# Autodesk Inventor assembly: arm
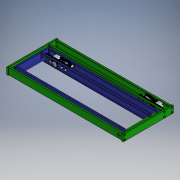
[picture p0: Inventor's stored thumbnail of the model, 180x180]
Saved by Autodesk Inventor 2022 (Build 260153000, 153)
## iProperties
Created: 2021-06-08
Part Number: arm
Document SubType Name: Assembly
Designer: yossy
Mass: 1577.87 g
Surface Area: 2797.55 cm^2
Volume: 584.398 cm^3
Density: 2.7 g/cm^3
Author: yossy
## Documents named in this file (21)
- C:\Users\nrz71\Documents\Inventor\arm\arm.iam
- C:\Users\nrz71\Documents\Inventor\arm\arm1_L.ipt
- C:\Users\nrz71\Documents\Inventor\arm\arm1_S.ipt
- C:\Users\nrz71\Documents\Inventor\arm\arm1_L_hole.ipt
- C:\Users\nrz71\Documents\Inventor\arm\arm1_L_M.ipt
- C:\Users\nrz71\Documents\Inventor\arm\110041_AMAX16_EB_2W_SL_1WE.ipt
- C:\Users\nrz71\Downloads\PARTserver0202107062223180363888451784290\BS2M30.ipt
- C:\Users\nrz71\Documents\Inventor\arm\arm\デザイン アクセラレータ\平歯車3.iam
- C:\Users\nrz71\Documents\Inventor\arm\軸.ipt
- C:\Users\nrz71\Downloads\BS2M14_Autodesk_Inventor_2020_20210707\BS2M14.ipt
- C:\Users\nrz71\Documents\Inventor\arm\arm\デザイン アクセラレータ\平歯車6.iam
- C:\Users\nrz71\Documents\Inventor\arm\大軸.ipt
- C:\Users\nrz71\Documents\Inventor\arm\arm1_L - コピー.ipt
- C:\Users\nrz71\Documents\Inventor\arm\arm1_L_hole - コピー.ipt
- C:\Users\nrz71\Documents\Inventor\arm\arm1_S - コピー.ipt
- C:\Users\nrz71\Documents\Inventor\arm\arm1_L_M - コピー.ipt
- C:\Users\nrz71\Documents\Inventor\arm\中軸.ipt
- C:\Users\nrz71\Documents\Inventor\arm\ベアリング\ベアリング4-7.ipt
- C:\Users\nrz71\Documents\Inventor\arm\ベアリング\ベアリング6-10.ipt
- C:\Users\nrz71\Documents\Inventor\arm\s2m187.ipt
- C:\Users\nrz71\Documents\Inventor\arm\s2m88.ipt
## Components (53 placed, 19 different names)
1. arm1_L:1 — メイト:1, メイト:2, フラッシュ:1, フラッシュ:3, フラッシュ:4, 正接:1, メイト:6, メイト:7, フラッシュ:6, メイト:24, メイト:25, フラッシュ:8, フラッシュ:18, メイト:45, メイト:59, メイト:61, メイト:62, メイト:65, メイト:71, メイト:115
2. arm1_S:1 — メイト:1, メイト:2, フラッシュ:1, メイト:3, フラッシュ:2, メイト:4, フラッシュ:5
3. arm1_L_hole:1 — フラッシュ:3, フラッシュ:4, メイト:5, メイト:10, メイト:11, メイト:13, メイト:17, メイト:22, メイト:23, メイト:27, メイト:28, メイト:29, メイト:31, メイト:32, メイト:39, メイト:47, メイト:48, メイト:58, メイト:63, メイト:64, メイト:70, フラッシュ:24, フラッシュ:25
4. arm1_L_M:1 — メイト:3, フラッシュ:2, メイト:4, メイト:68
5. 110041_AMAX16_EB_2W_SL_1WE:1 — メイト:5, 正接:1, メイト:6, メイト:13, メイト:21
6. arm1_S:2 — フラッシュ:5, メイト:7, フラッシュ:6
7. BS2M30:1 — メイト:10, メイト:11
8. 軸:1 — メイト:17, メイト:20, フラッシュ:18, メイト:57, メイト:60, メイト:116
9. BS2M30:2 — メイト:24, メイト:26, メイト:27
10. BS2M14:1 — メイト:20, メイト:25
11. 平歯車:1 [sub-assembly] — メイト:21, メイト:22, メイト:23
12. 平歯車:2 [sub-assembly] — メイト:26, メイト:28, メイト:30
13. BS2M30:3 — メイト:29, メイト:30, メイト:31
14. 大軸:1 — フラッシュ:8, メイト:32, メイト:33, メイト:66, メイト:67, メイト:69
15. arm1_L - コピー:1 — メイト:33, メイト:34, フラッシュ:10, メイト:35, フラッシュ:11, メイト:37, フラッシュ:12, メイト:38, フラッシュ:16, メイト:42, メイト:49, メイト:50, メイト:55, メイト:56, メイト:75, メイト:80, メイト:81, フラッシュ:22, メイト:90, メイト:97, フラッシュ:24, メイト:114
16. arm1_L_hole - コピー:1 — メイト:34, フラッシュ:10, メイト:36, メイト:51, メイト:52, メイト:53, メイト:54, メイト:77, メイト:78, メイト:79, メイト:99, メイト:110
17. 110041_AMAX16_EB_2W_SL_1WE:2 — メイト:35, フラッシュ:11, メイト:36, メイト:100
18. arm1_S - コピー:1 — メイト:37, フラッシュ:12, メイト:38, メイト:39, メイト:40, メイト:41, フラッシュ:13
19. arm1_L_M - コピー:1 — メイト:40, メイト:41, フラッシュ:13, メイト:72
20. 中軸:1 — フラッシュ:16, メイト:42, メイト:73, メイト:74, メイト:76, メイト:87, メイト:111
21. ベアリング4-7:2 — メイト:59, メイト:60
22. ベアリング4-7:3 — メイト:45, メイト:71, メイト:82, フラッシュ:19
23. ベアリング4-7:4 — メイト:47, メイト:48
24. ベアリング4-7:6 — メイト:49, メイト:50
25. ベアリング4-7:7 — メイト:55, メイト:56, フラッシュ:21
26. ベアリング4-7:8 — メイト:53, メイト:54, メイト:86
27. ベアリング4-7:9 — メイト:51, メイト:52, メイト:85
28. ベアリング4-7:10 — メイト:57, メイト:58
29. ベアリング6-10:1 — メイト:65, メイト:66
30. ベアリング6-10:2 — メイト:67, メイト:68
31. ベアリング6-10:3 — メイト:74, メイト:75
32. ベアリング6-10:4 — メイト:72, メイト:73
33. ベアリング4-7:11 — メイト:63, メイト:64
34. ベアリング4-7:12 — メイト:61, メイト:62, メイト:83, フラッシュ:20
35. ベアリング6-10:5 — メイト:69, メイト:70
36. ベアリング6-10:6 — メイト:76, メイト:77, メイト:92
37. ベアリング4-7:13 — メイト:80, メイト:81, フラッシュ:23
38. ベアリング4-7:14 — メイト:78, メイト:79, メイト:84, メイト:91
39. 軸:2 — メイト:82, フラッシュ:19, メイト:117
40. 軸:3 — メイト:83, フラッシュ:20
41. 軸:4 — メイト:86, フラッシュ:21, メイト:96, メイト:98, メイト:112
42. 軸:5 — メイト:85, フラッシュ:22, メイト:89, メイト:95, メイト:113
43. 軸:6 — メイト:84, フラッシュ:23, メイト:88, メイト:94, メイト:109
44. BS2M30:4 — メイト:87, メイト:92
45. BS2M30:5 — メイト:89, メイト:90
46. BS2M30:6 — メイト:88, メイト:91, メイト:93
47. 平歯車:3 [sub-assembly] — メイト:93, メイト:94, メイト:95
48. BS2M14:2 — メイト:96, メイト:97
49. 平歯車:4 [sub-assembly] — メイト:98, メイト:99, メイト:100
50. s2m187:1 — フラッシュ:25
51. s2m187:2 — メイト:109, メイト:110, メイト:111
52. s2m88:1 — メイト:112, メイト:113, メイト:114
53. s2m88:2 — メイト:115, メイト:116, メイト:117
## Relationships (119: Mate 98, Flush 20, Tangent 1)
- メイト:1 [Mate]: arm1_L:1 ↔ arm1_S:1
- メイト:2 [Mate]: arm1_L:1 ↔ arm1_S:1
- フラッシュ:1 [Flush]: arm1_L:1 ↔ arm1_S:1
- メイト:3 [Mate]: arm1_S:1 ↔ arm1_L_M:1
- フラッシュ:2 [Flush]: arm1_S:1 ↔ arm1_L_M:1
- メイト:4 [Mate]: arm1_S:1 ↔ arm1_L_M:1
- フラッシュ:3 [Flush]: arm1_L:1 ↔ arm1_L_hole:1
- フラッシュ:4 [Flush]: arm1_L:1 ↔ arm1_L_hole:1
- メイト:5 [Mate]: arm1_L_hole:1 ↔ 110041_AMAX16_EB_2W_SL_1WE:1
- 正接:1 [Tangent]: arm1_L:1 ↔ 110041_AMAX16_EB_2W_SL_1WE:1
- メイト:6 [Mate]: arm1_L:1 ↔ 110041_AMAX16_EB_2W_SL_1WE:1
- フラッシュ:5 [Flush]: arm1_S:1 ↔ arm1_S:2
- メイト:7 [Mate]: arm1_L:1 ↔ arm1_S:2
- フラッシュ:6 [Flush]: arm1_L:1 ↔ arm1_S:2
- メイト:10 [Mate]: arm1_L_hole:1 ↔ BS2M30:1
- メイト:11 [Mate]: arm1_L_hole:1 ↔ BS2M30:1
- メイト:13 [Mate]: arm1_L_hole:1 ↔ 110041_AMAX16_EB_2W_SL_1WE:1
- メイト:17 [Mate]: arm1_L_hole:1 ↔ 軸:1
- メイト:20 [Mate]: 軸:1 ↔ BS2M14:1
- メイト:21 [Mate]: 110041_AMAX16_EB_2W_SL_1WE:1 ↔ 平歯車:1
- メイト:22 [Mate]: arm1_L_hole:1 ↔ 平歯車:1
- メイト:23 [Mate]: arm1_L_hole:1 ↔ 平歯車:1
- メイト:24 [Mate]: arm1_L:1 ↔ BS2M30:2
- メイト:25 [Mate]: arm1_L:1 ↔ BS2M14:1
- メイト:26 [Mate]: BS2M30:2 ↔ 平歯車:2
- メイト:27 [Mate]: arm1_L_hole:1 ↔ BS2M30:2
- メイト:28 [Mate]: arm1_L_hole:1 ↔ 平歯車:2
- メイト:29 [Mate]: arm1_L_hole:1 ↔ BS2M30:3
- メイト:30 [Mate]: 平歯車:2 ↔ BS2M30:3
- メイト:31 [Mate]: arm1_L_hole:1 ↔ BS2M30:3
- フラッシュ:8 [Flush]: arm1_L:1 ↔ 大軸:1
- メイト:32 [Mate]: arm1_L_hole:1 ↔ 大軸:1
- メイト:33 [Mate]: 大軸:1 ↔ arm1_L - コピー:1
- メイト:34 [Mate]: arm1_L - コピー:1 ↔ arm1_L_hole - コピー:1
- フラッシュ:10 [Flush]: arm1_L - コピー:1 ↔ arm1_L_hole - コピー:1
- メイト:35 [Mate]: arm1_L - コピー:1 ↔ 110041_AMAX16_EB_2W_SL_1WE:2
- フラッシュ:11 [Flush]: arm1_L - コピー:1 ↔ 110041_AMAX16_EB_2W_SL_1WE:2
- メイト:36 [Mate]: arm1_L_hole - コピー:1 ↔ 110041_AMAX16_EB_2W_SL_1WE:2
- メイト:37 [Mate]: arm1_L - コピー:1 ↔ arm1_S - コピー:1
- フラッシュ:12 [Flush]: arm1_L - コピー:1 ↔ arm1_S - コピー:1
- メイト:38 [Mate]: arm1_L - コピー:1 ↔ arm1_S - コピー:1
- メイト:39 [Mate] (3 mm): arm1_L_hole:1 ↔ arm1_S - コピー:1
- メイト:40 [Mate]: arm1_S - コピー:1 ↔ arm1_L_M - コピー:1
- メイト:41 [Mate]: arm1_S - コピー:1 ↔ arm1_L_M - コピー:1
- フラッシュ:13 [Flush]: arm1_S - コピー:1 ↔ arm1_L_M - コピー:1
- フラッシュ:16 [Flush]: arm1_L - コピー:1 ↔ 中軸:1
- メイト:42 [Mate]: arm1_L - コピー:1 ↔ 中軸:1
- フラッシュ:18 [Flush]: arm1_L:1 ↔ 軸:1
- メイト:45 [Mate]: arm1_L:1 ↔ ベアリング4-7:3
- メイト:47 [Mate]: arm1_L_hole:1 ↔ ベアリング4-7:4
- メイト:48 [Mate]: arm1_L_hole:1 ↔ ベアリング4-7:4
- メイト:49 [Mate]: arm1_L - コピー:1 ↔ ベアリング4-7:6
- メイト:50 [Mate]: arm1_L - コピー:1 ↔ ベアリング4-7:6
- メイト:51 [Mate]: arm1_L_hole - コピー:1 ↔ ベアリング4-7:9
- メイト:52 [Mate]: arm1_L_hole - コピー:1 ↔ ベアリング4-7:9
- メイト:53 [Mate]: arm1_L_hole - コピー:1 ↔ ベアリング4-7:8
- メイト:54 [Mate]: arm1_L_hole - コピー:1 ↔ ベアリング4-7:8
- メイト:55 [Mate]: arm1_L - コピー:1 ↔ ベアリング4-7:7
- メイト:56 [Mate]: arm1_L - コピー:1 ↔ ベアリング4-7:7
- メイト:57 [Mate]: 軸:1 ↔ ベアリング4-7:10
- メイト:58 [Mate]: arm1_L_hole:1 ↔ ベアリング4-7:10
- メイト:59 [Mate]: arm1_L:1 ↔ ベアリング4-7:2
- メイト:60 [Mate]: 軸:1 ↔ ベアリング4-7:2
- メイト:61 [Mate]: arm1_L:1 ↔ ベアリング4-7:12
- メイト:62 [Mate]: arm1_L:1 ↔ ベアリング4-7:12
- メイト:63 [Mate]: arm1_L_hole:1 ↔ ベアリング4-7:11
- メイト:64 [Mate]: arm1_L_hole:1 ↔ ベアリング4-7:11
- メイト:65 [Mate]: arm1_L:1 ↔ ベアリング6-10:1
- メイト:66 [Mate]: 大軸:1 ↔ ベアリング6-10:1
- メイト:67 [Mate]: 大軸:1 ↔ ベアリング6-10:2
- メイト:68 [Mate]: arm1_L_M:1 ↔ ベアリング6-10:2
- メイト:69 [Mate]: 大軸:1 ↔ ベアリング6-10:5
- メイト:70 [Mate]: arm1_L_hole:1 ↔ ベアリング6-10:5
- メイト:71 [Mate]: arm1_L:1 ↔ ベアリング4-7:3
- メイト:72 [Mate]: arm1_L_M - コピー:1 ↔ ベアリング6-10:4
- メイト:73 [Mate]: 中軸:1 ↔ ベアリング6-10:4
- メイト:74 [Mate]: 中軸:1 ↔ ベアリング6-10:3
- メイト:75 [Mate]: arm1_L - コピー:1 ↔ ベアリング6-10:3
- メイト:76 [Mate]: 中軸:1 ↔ ベアリング6-10:6
- メイト:77 [Mate]: arm1_L_hole - コピー:1 ↔ ベアリング6-10:6
- メイト:78 [Mate]: arm1_L_hole - コピー:1 ↔ ベアリング4-7:14
- メイト:79 [Mate]: arm1_L_hole - コピー:1 ↔ ベアリング4-7:14
- メイト:80 [Mate]: arm1_L - コピー:1 ↔ ベアリング4-7:13
- メイト:81 [Mate]: arm1_L - コピー:1 ↔ ベアリング4-7:13
- メイト:82 [Mate]: ベアリング4-7:3 ↔ 軸:2
- フラッシュ:19 [Flush]: ベアリング4-7:3 ↔ 軸:2
- メイト:83 [Mate]: ベアリング4-7:12 ↔ 軸:3
- フラッシュ:20 [Flush]: ベアリング4-7:12 ↔ 軸:3
- メイト:84 [Mate]: ベアリング4-7:14 ↔ 軸:6
- メイト:85 [Mate]: ベアリング4-7:9 ↔ 軸:5
- メイト:86 [Mate]: ベアリング4-7:8 ↔ 軸:4
- フラッシュ:21 [Flush]: ベアリング4-7:7 ↔ 軸:4
- フラッシュ:22 [Flush]: arm1_L - コピー:1 ↔ 軸:5
- フラッシュ:23 [Flush]: ベアリング4-7:13 ↔ 軸:6
- メイト:87 [Mate]: 中軸:1 ↔ BS2M30:4
- メイト:88 [Mate]: 軸:6 ↔ BS2M30:6
- メイト:89 [Mate]: 軸:5 ↔ BS2M30:5
- メイト:90 [Mate]: arm1_L - コピー:1 ↔ BS2M30:5
- メイト:91 [Mate]: ベアリング4-7:14 ↔ BS2M30:6
- メイト:92 [Mate]: ベアリング6-10:6 ↔ BS2M30:4
- メイト:93 [Mate]: BS2M30:6 ↔ 平歯車:3
- メイト:94 [Mate]: 軸:6 ↔ 平歯車:3
- メイト:95 [Mate]: 軸:5 ↔ 平歯車:3
- メイト:96 [Mate]: 軸:4 ↔ BS2M14:2
- メイト:97 [Mate]: arm1_L - コピー:1 ↔ BS2M14:2
- メイト:98 [Mate]: 軸:4 ↔ 平歯車:4
- メイト:99 [Mate]: arm1_L_hole - コピー:1 ↔ 平歯車:4
- メイト:100 [Mate]: 110041_AMAX16_EB_2W_SL_1WE:2 ↔ 平歯車:4
- フラッシュ:24 [Flush]: arm1_L_hole:1 ↔ arm1_L - コピー:1
- フラッシュ:25 [Flush]: arm1_L_hole:1 ↔ s2m187:1
- メイト:109 [Mate]: 軸:6 ↔ s2m187:2
- メイト:110 [Mate]: arm1_L_hole - コピー:1 ↔ s2m187:2
- メイト:111 [Mate]: 中軸:1 ↔ s2m187:2
- メイト:112 [Mate]: 軸:4 ↔ s2m88:1
- メイト:113 [Mate]: 軸:5 ↔ s2m88:1
- メイト:114 [Mate]: arm1_L - コピー:1 ↔ s2m88:1
- メイト:115 [Mate]: arm1_L:1 ↔ s2m88:2
- メイト:116 [Mate]: 軸:1 ↔ s2m88:2
- メイト:117 [Mate]: 軸:2 ↔ s2m88:2
